# Autodesk Inventor assembly: Assembly
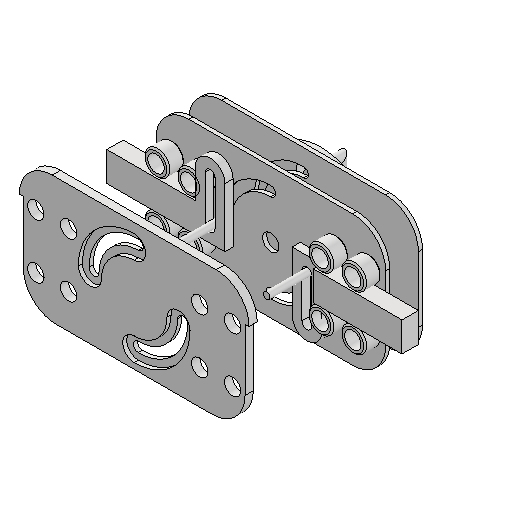
[picture p0: Inventor's stored thumbnail of the model, 512x512]
Saved by Autodesk Inventor 2025 (Build 290162000, 162)
## iProperties
Created: 2024-02-12
Part Number: Assembly
Document SubType Name: Assembly
Designer: calvi
Author: calvi
## Documents named in this file (11)
- C:\Users\seene\Desktop\Stony Brook\SBRT\RCR_Dexter\Chassis\Battery Drawer\Assembly.iam
- C:\Users\seene\Desktop\Stony Brook\SBRT\RCR_Dexter\Chassis\Battery Drawer\Plate.ipt
- C:\Users\seene\Desktop\Stony Brook\SBRT\RCR_Dexter\Chassis\Battery Drawer\Crank.ipt
- C:\Users\seene\Desktop\Stony Brook\SBRT\RCR_Dexter\Chassis\Battery Drawer\Handle.ipt
- C:\Users\seene\Desktop\Stony Brook\SBRT\RCR_Dexter\Chassis\Battery Drawer\Front_plate.ipt
- C:\Users\seene\Desktop\Stony Brook\SBRT\RCR_Dexter\Chassis\Battery Drawer\6389K345_Light Duty Dry-Running Nylon Sleeve Bearing\6389K345_Light Duty Dry-Running Nylon Sleeve Bearing.ipt
- C:\Users\seene\Desktop\Stony Brook\SBRT\RCR_Dexter\Chassis\Battery Drawer\Slider1.ipt
- Slider1.ipt
- C:\Users\seene\Desktop\Stony Brook\SBRT\RCR_Dexter\Chassis\Battery Drawer\Slider2.ipt
- C:\Users\seene\Desktop\Stony Brook\SBRT\RCR_Dexter\Chassis\Battery Drawer\Peg.ipt
- C:\Users\seene\Desktop\Stony Brook\SBRT\RCR_Dexter\Chassis\Battery Drawer\Back_plate.ipt
## Components (17 placed, 9 different names)
1. Plate:1 — Rigid:1, Rotational:2, Rotational:3, Rotational:4, Rotational:5, Rotational:6, Rotational:7, Rotational:8, Rotational:9, Mate:1, Mate:2, Mate:3, Mate:4
2. Crank:1 — Rotational:1, Mate:5, Mate:6, Cylindrical:2, Cylindrical:3
3. Handle:1 — Mate:5, Mate:6
4. Front_plate:1 — Rotational:1, Rigid:1
5. Slider1:1 — Mate:1, Mate:2, Slider:2
6. Slider2:1 — Mate:3, Mate:4, Slider:1
7. Peg:1 — Slider:1, Cylindrical:3
8. Peg:2 — Cylindrical:2, Slider:2
9. Back_plate:1 — Rotational:10, Rotational:11
10. 6389K345_Light Duty Dry-Running Nylon Sleeve Bearing:8 — Rotational:7
11. 6389K345_Light Duty Dry-Running Nylon Sleeve Bearing:7 — Rotational:9
12. 6389K345_Light Duty Dry-Running Nylon Sleeve Bearing:6 — Rotational:6
13. 6389K345_Light Duty Dry-Running Nylon Sleeve Bearing:5 — Rotational:8
14. 6389K345_Light Duty Dry-Running Nylon Sleeve Bearing:4 — Rotational:5
15. 6389K345_Light Duty Dry-Running Nylon Sleeve Bearing:3 — Rotational:4, Rotational:11
16. 6389K345_Light Duty Dry-Running Nylon Sleeve Bearing:2 — Rotational:2
17. 6389K345_Light Duty Dry-Running Nylon Sleeve Bearing:1 — Rotational:3, Rotational:10
## Relationships (22: RevoluteJoint 11, Mate 6, CylindricalJoint 2, TranslationJoint 2, WeldJoint 1)
- Rotational:1 [RevoluteJoint]: Crank:1 ↔ Front_plate:1
- Rigid:1 [WeldJoint] (-22.225 mm): Plate:1 ↔ Front_plate:1
- Rotational:2 [RevoluteJoint]: Plate:1 ↔ 6389K345_Light Duty Dry-Running Nylon Sleeve Bearing:2
- Rotational:3 [RevoluteJoint]: Plate:1 ↔ 6389K345_Light Duty Dry-Running Nylon Sleeve Bearing:1
- Rotational:4 [RevoluteJoint]: Plate:1 ↔ 6389K345_Light Duty Dry-Running Nylon Sleeve Bearing:3
- Rotational:5 [RevoluteJoint]: Plate:1 ↔ 6389K345_Light Duty Dry-Running Nylon Sleeve Bearing:4
- Rotational:6 [RevoluteJoint]: Plate:1 ↔ 6389K345_Light Duty Dry-Running Nylon Sleeve Bearing:6
- Rotational:7 [RevoluteJoint]: Plate:1 ↔ 6389K345_Light Duty Dry-Running Nylon Sleeve Bearing:8
- Rotational:8 [RevoluteJoint]: Plate:1 ↔ 6389K345_Light Duty Dry-Running Nylon Sleeve Bearing:5
- Rotational:9 [RevoluteJoint]: Plate:1 ↔ 6389K345_Light Duty Dry-Running Nylon Sleeve Bearing:7
- Mate:1: Plate:1 ↔ Slider1:1
- Mate:2 (-11.43 mm): Plate:1 ↔ Slider1:1
- Mate:3: Plate:1 ↔ Slider2:1
- Mate:4 (-11.43 mm): Plate:1 ↔ Slider2:1
- Mate:5: Crank:1 ↔ Handle:1
- Mate:6: Crank:1 ↔ Handle:1
- Cylindrical:2: Crank:1 ↔ Peg:2
- Slider:1 [TranslationJoint]: Slider2:1 ↔ Peg:1
- Cylindrical:3: Crank:1 ↔ Peg:1
- Slider:2 [TranslationJoint]: Slider1:1 ↔ Peg:2
- Rotational:10 [RevoluteJoint]: Back_plate:1 ↔ 6389K345_Light Duty Dry-Running Nylon Sleeve Bearing:1
- Rotational:11 [RevoluteJoint]: Back_plate:1 ↔ 6389K345_Light Duty Dry-Running Nylon Sleeve Bearing:3
